# Autodesk Inventor assembly: pitch-frame
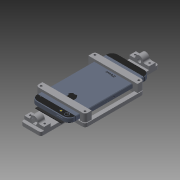
[picture p0: Inventor's stored thumbnail of the model, 180x180]
Saved by Autodesk Inventor 2015 (Build 190159000, 159)
## iProperties
Created: 2015-12-01
Part Number: pitch-frame
Document SubType Name: Assembly
Designer: jufranz
Author: jufranz
## Documents named in this file (6)
- \\engin-labs.m.storage.umich.edu\jufranz\windat.V2\Documents\Inventor\perspection\pitch-frame.iam
- \\engin-labs.m.storage.umich.edu\jufranz\windat.V2\Documents\Inventor\perspection\phone_plate.ipt
- \\engin-labs.m.storage.umich.edu\jufranz\windat.V2\Documents\Inventor\perspection\motor_bracket.ipt
- \\engin-labs.m.storage.umich.edu\jufranz\windat.V2\Documents\Inventor\perspection\apple-iphone-5-7.snapshot.1\iPhone 5 (Black).iam
- \\engin-labs.m.storage.umich.edu\jufranz\windat.V2\Documents\Inventor\perspection\phone_cushion.ipt
- \\engin-labs.m.storage.umich.edu\jufranz\windat.V2\Documents\Inventor\perspection\phone_clamp.ipt
## Components (7 placed, 5 different names)
1. phone_plate:1 — Insert:1, Insert:2, Insert:3, Insert:4, Mate:1, Insert:5, Insert:6, Insert:7, Insert:8
2. motor_bracket:1 — Insert:1, Insert:2
3. motor_bracket:2 — Insert:3, Insert:4
4. iPhone 5 (Black):1 [sub-assembly] — Mate:2
5. phone_cushion:1 — Mate:1, Mate:2
6. phone_clamp:1 — Insert:7, Insert:8
7. phone_clamp:2 — Insert:5, Insert:6
## Relationships (10: Insert 8, Mate 2)
- Insert:1: phone_plate:1 ↔ motor_bracket:1
- Insert:2: phone_plate:1 ↔ motor_bracket:1
- Insert:3: phone_plate:1 ↔ motor_bracket:2
- Insert:4: phone_plate:1 ↔ motor_bracket:2
- Mate:1: phone_plate:1 ↔ phone_cushion:1
- Mate:2: iPhone 5 (Black):1 ↔ phone_cushion:1
- Insert:5 (1 mm): phone_plate:1 ↔ phone_clamp:2
- Insert:6 (1 mm): phone_plate:1 ↔ phone_clamp:2
- Insert:7 (1 mm): phone_plate:1 ↔ phone_clamp:1
- Insert:8 (1 mm): phone_plate:1 ↔ phone_clamp:1
